# Autodesk Inventor assembly: Left Back Drive Wheel Assembly
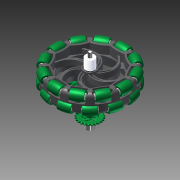
[picture p0: Inventor's stored thumbnail of the model, 180x180]
Saved by Autodesk Inventor 2012 (Build 160160000, 160)
## iProperties
Created: 2011-09-10
Part Number: Left Back Drive Wheel Assembly
Document SubType Name: Assembly
Designer: Wade
Author: Wade
## Documents named in this file (9)
- C:\Users\Wade\Documents\1103 Robot - CAD Assembly\Left Back Drive Wheel Assembly.iam
- C:\Users\Wade\Documents\1103 Robot - CAD Assembly\18 Tooth HS Sprocket.ipt
- C:\Users\Wade\Documents\24C VEX CAD Files\Wheels\4'' Omni-Directional Wheel.iam
- C:\Users\Wade\Documents\24C VEX CAD Files\Washers & Spacers\Spacer (Nylon), 0.500''.ipt
- C:\Users\Wade\Documents\24C VEX CAD Files\Washers & Spacers\Washer, Delrin.ipt
- C:\Users\Wade\Documents\24C VEX CAD Files\Other Parts\Shaft Collar (with Set Screw Installed).ipt
- C:\Users\Wade\Documents\24C VEX CAD Files\Drive Shafts\Drive Shaft (Square Bar) 3.625''.ipt
- C:\Users\Wade\Documents\24C VEX CAD Files\Washers & Spacers\Spacer (Nylon), 0.125''.ipt
- C:\Users\Wade\Documents\24C VEX CAD Files\Gears & Pulleys\24-Tooth Sprocket.ipt
## Components (9 placed, 8 different names)
1. 18 Tooth HS Sprocket:1 — Flush:1, Flush:3, Mate:5, Mate:6, Mate:7, Mate:10
2. 4'' Omni-Directional Wheel:1 [sub-assembly] — Mate:1, Mate:2, Flush:1, Mate:3, Mate:4, Flush:2, Flush:3
3. Spacer (Nylon), 0.500'':1 — Mate:1, Mate:2
4. Washer, Delrin:1 — Mate:6, Mate:7, Mate:11
5. Shaft Collar (with Set Screw Installed):1 — Mate:3, Mate:4, Flush:2, Mate:5
6. Drive Shaft (Square Bar) 3.625'':1 — Mate:14, Flush:5
7. Spacer (Nylon), 0.125'':1 — Mate:10, Mate:11, Mate:12, Mate:13
8. 24-Tooth Sprocket:1 — Mate:12, Mate:13, Mate:14, Mate:15, Mate:16
9. Shaft Collar (with Set Screw Installed):2 — Mate:15, Mate:16, Flush:5
## Relationships (21: Mate 16, Flush 5)
- Mate:1: 4'' Omni-Directional Wheel:1 ↔ Spacer (Nylon), 0.500'':1
- Mate:2: 4'' Omni-Directional Wheel:1 ↔ Spacer (Nylon), 0.500'':1
- Flush:1: 18 Tooth HS Sprocket:1 ↔ 4'' Omni-Directional Wheel:1
- Mate:3: 4'' Omni-Directional Wheel:1 ↔ Shaft Collar (with Set Screw Installed):1
- Mate:4: 4'' Omni-Directional Wheel:1 ↔ Shaft Collar (with Set Screw Installed):1
- Flush:2: 4'' Omni-Directional Wheel:1 ↔ Shaft Collar (with Set Screw Installed):1
- Flush:3: 18 Tooth HS Sprocket:1 ↔ 4'' Omni-Directional Wheel:1
- Mate:5: 18 Tooth HS Sprocket:1 ↔ Shaft Collar (with Set Screw Installed):1
- Mate:6: 18 Tooth HS Sprocket:1 ↔ Washer, Delrin:1
- Mate:7: 18 Tooth HS Sprocket:1 ↔ Washer, Delrin:1
- [Mate]: 18 Tooth HS Sprocket:1 ↔ Drive Shaft (Square Bar) 3.625'':1
- [Mate]: 18 Tooth HS Sprocket:1 ↔ Drive Shaft (Square Bar) 3.625'':1
- [Flush] (-6.35 mm): Spacer (Nylon), 0.500'':1 ↔ Drive Shaft (Square Bar) 3.625'':1
- Mate:10: 18 Tooth HS Sprocket:1 ↔ Spacer (Nylon), 0.125'':1
- Mate:11 (7.5184 mm): Washer, Delrin:1 ↔ Spacer (Nylon), 0.125'':1
- Mate:12: Spacer (Nylon), 0.125'':1 ↔ 24-Tooth Sprocket:1
- Mate:13: Spacer (Nylon), 0.125'':1 ↔ 24-Tooth Sprocket:1
- Mate:14: Drive Shaft (Square Bar) 3.625'':1 ↔ 24-Tooth Sprocket:1
- Mate:15: 24-Tooth Sprocket:1 ↔ Shaft Collar (with Set Screw Installed):2
- Mate:16: 24-Tooth Sprocket:1 ↔ Shaft Collar (with Set Screw Installed):2
- Flush:5: Drive Shaft (Square Bar) 3.625'':1 ↔ Shaft Collar (with Set Screw Installed):2
